# Autodesk Inventor assembly: 10-SUSP-ARM-02
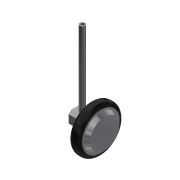
[picture p0: Inventor's stored thumbnail of the model, 180x180]
Saved by Autodesk Inventor 2018 (Build 220112000, 112)
## iProperties
Created: 2017-07-23
Part Number: 10-SUSP-ARM-02
Document SubType Name: Assembly
Designer: Martin Fees
Author: Martin Fees
## Documents named in this file (4)
- C:\Users\Martin Fees\Documents\NRBDL\Inventor-NRBDL\10-SUSP\10-SUSP-ARM-02.iam
- C:\Users\Martin Fees\Documents\NRBDL\Inventor-NRBDL\10-SUSP\10-004-ACTR-FIX.ipt
- C:\Users\Martin Fees\Documents\NRBDL\Inventor-NRBDL\10-SUSP\10-001-ACTR.ipt
- C:\Users\Martin Fees\Documents\NRBDL\Inventor-NRBDL\10-SUSP\10-005-PIPE.ipt
## Components (3 placed, 3 different names)
1. 10-004-ACTR-FIX:1 — Mate:1, Flush:1, Flush:2, Mate:2, Angle:1, Mate:3, Mate:4, Mate:5
2. 10-001-ACTR:1 — Mate:2, Angle:1, Mate:3
3. 10-005-PIPE:1 — Mate:4, Mate:5
## Relationships (8: Mate 5, Flush 2, Angle 1)
- Mate:1: 10-004-ACTR-FIX:1
- Flush:1: 10-004-ACTR-FIX:1
- Flush:2: 10-004-ACTR-FIX:1
- Mate:2: 10-004-ACTR-FIX:1 ↔ 10-001-ACTR:1
- Angle:1 (0 deg): 10-004-ACTR-FIX:1 ↔ 10-001-ACTR:1
- Mate:3: 10-004-ACTR-FIX:1 ↔ 10-001-ACTR:1
- Mate:4: 10-004-ACTR-FIX:1 ↔ 10-005-PIPE:1
- Mate:5: 10-004-ACTR-FIX:1 ↔ 10-005-PIPE:1
